# Autodesk Inventor assembly: FinalRobot-ver10-1111-2021
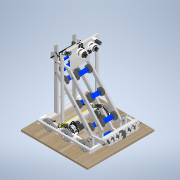
[picture p0: Inventor's stored thumbnail of the model, 180x180]
Saved by Autodesk Inventor 2021 (Build 250183000, 183)
## iProperties
Created: 2021-01-26
Part Number: FinalRobot-ver10-1111-2021
Document SubType Name: Assembly
Designer: Caitlin
Author: Caitlin
## Documents named in this file (5)
- E:\PHRC CADD 2021\PHRC CADD\2020 Infinite Recharge\2021 Infinite Recharge\FinalRobot-ver10-1111-2021.iam
- E:\PHRC CADD 2021\PHRC CADD\2020 Infinite Recharge\2021 Infinite Recharge\Chassis\Chassis-ver1-1111-2021.iam
- E:\PHRC CADD 2021\PHRC CADD\2020 Infinite Recharge\Platform.ver1-1111-2020.ipt
- E:\PHRC CADD 2021\PHRC CADD\2020 Infinite Recharge\2021 Infinite Recharge\Chassis\Shooter-Storage-IntakeAssembly.ver4-1111-2021.iam
- E:\PHRC CADD 2021\PHRC CADD\2020 Infinite Recharge\2021 Infinite Recharge\Chassis\PnumaticActiveClimb-ver3-1111-2021.iam
## Components (4 placed, 4 different names)
1. Chassis-ver1-1111-2021:1 [sub-assembly] — Mate:1, Angle:1, Flush:1, Flush:2, Mate:2, Mate:3, Flush:3, Mate:4, Flush:4, Flush:5
2. Platform.ver1-1111-2020:1 — Mate:1, Angle:1, Flush:1, Flush:2
3. Shooter-Storage-IntakeAssembly.ver4-1111-2021:1 [sub-assembly] — Mate:2, Mate:3, Flush:3
4. PnumaticActiveClimb-ver3-1111-2021:1 [sub-assembly] — Mate:4, Flush:4, Flush:5
## Relationships (10: Flush 5, Mate 4, Angle 1)
- Mate:1 (47.625 mm): Chassis-ver1-1111-2021:1 ↔ Platform.ver1-1111-2020:1
- Angle:1 (0 deg): Chassis-ver1-1111-2021:1 ↔ Platform.ver1-1111-2020:1
- Flush:1 (152.4 mm): Chassis-ver1-1111-2021:1 ↔ Platform.ver1-1111-2020:1
- Flush:2 (114.3 mm): Chassis-ver1-1111-2021:1 ↔ Platform.ver1-1111-2020:1
- Mate:2: Chassis-ver1-1111-2021:1 ↔ Shooter-Storage-IntakeAssembly.ver4-1111-2021:1
- Mate:3: Chassis-ver1-1111-2021:1 ↔ Shooter-Storage-IntakeAssembly.ver4-1111-2021:1
- Flush:3: Chassis-ver1-1111-2021:1 ↔ Shooter-Storage-IntakeAssembly.ver4-1111-2021:1
- Mate:4: Chassis-ver1-1111-2021:1 ↔ PnumaticActiveClimb-ver3-1111-2021:1
- Flush:4: Chassis-ver1-1111-2021:1 ↔ PnumaticActiveClimb-ver3-1111-2021:1
- Flush:5: Chassis-ver1-1111-2021:1 ↔ PnumaticActiveClimb-ver3-1111-2021:1
